# Autodesk Inventor assembly: POM_T5_05
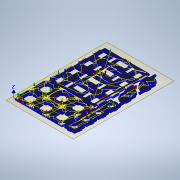
[picture p0: Inventor's stored thumbnail of the model, 180x180]
Saved by Autodesk Inventor 2020 (Build 240168000, 168)
## iProperties
Created: 2021-08-27
Part Number: POM_T5_05
Document SubType Name: Assembly
Designer: Masato
Author: Masato
## Documents named in this file (6)
- D:\GitHub\inventor\SUSTAINA-OP\Cam\POM_T5_05.iam
- D:\GitHub\inventor\SUSTAINA-OP\Cam\DisposableBoard.ipt
- D:\GitHub\inventor\SUSTAINA-OP\UpperBody\Head\Camera_root_frame_e-CAM50_CUNX.ipt
- D:\GitHub\inventor\SUSTAINA-OP\UpperBody\Arm\UpperArm_diagonal.ipt
- D:\GitHub\inventor\SUSTAINA-OP\UpperBody\Head\Camera_side_frame.ipt
- D:\GitHub\inventor\SUSTAINA-OP\UpperBody\Trunk\Trunk_chest_frame.ipt
## Components (19 placed, 5 different names)
1. DisposableBoard:1 — メイト:2, メイト:1, フラッシュ:1, フラッシュ:2, メイト:4, メイト:5, メイト:6, メイト:7, メイト:8, メイト:9, メイト:10, メイト:12, メイト:13, メイト:14, メイト:16, メイト:17, メイト:20, メイト:22, メイト:23
2. Camera_side_frame:1 — メイト:13, メイト:14, メイト:15, メイト:19
3. Camera_side_frame:4 — メイト:17, メイト:20, メイト:24
4. Camera_side_frame:5 — メイト:16, メイト:18, メイト:19
5. Camera_side_frame:6 — メイト:21, メイト:22, メイト:23, メイト:24
6. Camera_root_frame_e-CAM50_CUNX:1 — メイト:4, メイト:5, メイト:6
7. Camera_root_frame_e-CAM50_CUNX:2 — メイト:11
8. Camera_root_frame_e-CAM50_CUNX:3
9. Camera_root_frame_e-CAM50_CUNX:4
10. Camera_root_frame_e-CAM50_CUNX:5
11. Camera_root_frame_e-CAM50_CUNX:6
12. UpperArm_diagonal:1 — メイト:7, メイト:8, メイト:9
13. UpperArm_diagonal:2
14. UpperArm_diagonal:3
15. UpperArm_diagonal:4 — メイト:15
16. Trunk_chest_frame:1 — メイト:10, メイト:11, メイト:12
17. Trunk_chest_frame:2
18. Trunk_chest_frame:3 — メイト:18
19. Trunk_chest_frame:4 — メイト:21
## Component patterns: (6 elements, first: Camera_root_frame_e-CAM50_CUNX:1), (4 elements, first: UpperArm_diagonal:1), (4 elements, first: Trunk_chest_frame:1)
## Relationships (25: Mate 23, Flush 2)
- メイト:2 [Mate]: DisposableBoard:1
- メイト:1 [Mate]: DisposableBoard:1
- フラッシュ:1 [Flush]: DisposableBoard:1
- フラッシュ:2 [Flush]: DisposableBoard:1
- メイト:4 [Mate]: DisposableBoard:1 ↔ Camera_root_frame_e-CAM50_CUNX:1
- メイト:5 [Mate] (2 mm): DisposableBoard:1 ↔ Camera_root_frame_e-CAM50_CUNX:1
- メイト:6 [Mate] (2 mm): DisposableBoard:1 ↔ Camera_root_frame_e-CAM50_CUNX:1
- メイト:7 [Mate]: DisposableBoard:1 ↔ UpperArm_diagonal:1
- メイト:8 [Mate] (2 mm): DisposableBoard:1 ↔ UpperArm_diagonal:1
- メイト:9 [Mate] (2 mm): DisposableBoard:1 ↔ UpperArm_diagonal:1
- メイト:10 [Mate]: DisposableBoard:1 ↔ Trunk_chest_frame:1
- メイト:11 [Mate] (2.5 mm): Camera_root_frame_e-CAM50_CUNX:2 ↔ Trunk_chest_frame:1
- メイト:12 [Mate] (2 mm): DisposableBoard:1 ↔ Trunk_chest_frame:1
- メイト:13 [Mate]: DisposableBoard:1 ↔ Camera_side_frame:1
- メイト:14 [Mate] (5 mm): DisposableBoard:1 ↔ Camera_side_frame:1
- メイト:15 [Mate] (2.5 mm): Camera_side_frame:1 ↔ UpperArm_diagonal:4
- メイト:16 [Mate]: DisposableBoard:1 ↔ Camera_side_frame:5
- メイト:17 [Mate]: DisposableBoard:1 ↔ Camera_side_frame:4
- メイト:18 [Mate] (3 mm): Camera_side_frame:5 ↔ Trunk_chest_frame:3
- メイト:19 [Mate] (10 mm): Camera_side_frame:1 ↔ Camera_side_frame:5
- メイト:20 [Mate] (5 mm): DisposableBoard:1 ↔ Camera_side_frame:4
- メイト:21 [Mate] (3 mm): Camera_side_frame:6 ↔ Trunk_chest_frame:4
- メイト:22 [Mate]: DisposableBoard:1 ↔ Camera_side_frame:6
- メイト:23 [Mate] (2 mm): DisposableBoard:1 ↔ Camera_side_frame:6
- メイト:24 [Mate] (9 mm): Camera_side_frame:4 ↔ Camera_side_frame:6
